# Autodesk Inventor assembly: assembly_connector
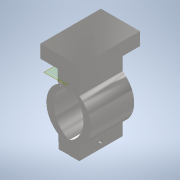
[picture p0: Inventor's stored thumbnail of the model, 180x180]
Saved by Autodesk Inventor 2021 (Build 250183000, 183)
## iProperties
Created: 2021-05-17
Part Number: assembly_connector
Document SubType Name: Assembly
Designer: chick
Author: chick
## Documents named in this file (9)
- C:\Users\chick\OneDrive - Flinders\Chi Ki Siu Work\CAD work\assembly_connector.iam
- C:\Users\chick\OneDrive - Flinders\Chi Ki Siu Work\CAD work\left_part.ipt
- C:\Users\chick\OneDrive - Flinders\Chi Ki Siu Work\CAD work\Hinge.ipt
- C:\Users\chick\OneDrive - Flinders\Chi Ki Siu Work\CAD work\assembly_connector\AIP\FEA\dm8i2qu8w.fins
- C:\Users\chick\OneDrive - Flinders\Chi Ki Siu Work\CAD work\assembly_connector\AIP\FEA\dm8i2qu8w.fsat
- C:\Users\chick\OneDrive - Flinders\Chi Ki Siu Work\CAD work\assembly_connector\AIP\FEA\dm8i2qu8w.ftes
- C:\Users\chick\OneDrive - Flinders\Chi Ki Siu Work\CAD work\assembly_connector\AIP\FEA\dm8i2qu8w.fwiz
- C:\Users\chick\OneDrive - Flinders\Chi Ki Siu Work\CAD work\assembly_connector\AIP\FEA\dm8i2qu9s.fmsh
- C:\Users\chick\OneDrive - Flinders\Chi Ki Siu Work\CAD work\assembly_connector\AIP\FEA\dm8i2qu9t.fres
## Components (2 placed, 2 different names)
1. left_part:1 — Mate:2, Mate:3
2. Hinge:1 — Mate:2, Mate:3
## Relationships (2: Mate 2)
- Mate:2: left_part:1 ↔ Hinge:1
- Mate:3: left_part:1 ↔ Hinge:1
## Named parameters: sa_0 = 49050, sa_1 = 10000
note: some values were not read from the file. Shown as the stored number, unit unknown: "sa_0", "sa_1".
